# Autodesk Inventor assembly: Dedao_Mecanismo_Posição2_ComDedao
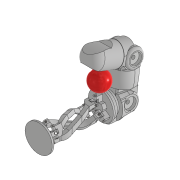
[picture p0: Inventor's stored thumbnail of the model, 180x180]
Saved by Autodesk Inventor 2020 (Build 240168000, 168)
## iProperties
Created: 2021-04-01
Part Number: Dedao_Mecanismo_Posição2_ComDedao
Document SubType Name: Assembly
Designer: deox
Author: deox
## Documents named in this file (11)
- C:\Users\deox\Desktop\TCC\Inventor Files\Dedo Kick\Dedao_Mecanismo_Posição2_ComDedao.iam
- C:\Users\deox\Desktop\TCC\Inventor Files\Dedo Kick\Base_Dedao.ipt
- C:\Users\deox\Desktop\TCC\Inventor Files\Dedo Kick\KNUCKLE_Dedao.ipt
- C:\Users\deox\Desktop\TCC\Inventor Files\Dedo Kick\LEG_Dedao.ipt
- C:\Users\deox\Desktop\TCC\Inventor Files\Dedo Kick\Pin_Dedao.ipt
- C:\Users\deox\Desktop\TCC\Inventor Files\Dedo Kick\Base_DEDAO_rot.ipt
- C:\Users\deox\Desktop\TCC\Inventor Files\Dedo Kick\Middle_DEDAO.ipt
- C:\Users\deox\Desktop\TCC\Inventor Files\Dedo Kick\ShameHider_DEDAO.ipt
- C:\Users\deox\Desktop\TCC\Inventor Files\Dedo Kick\Tip_DEDAO.ipt
- C:\Users\deox\Desktop\TCC\Inventor Files\Dedo Kick\TipTip_DEDAO.ipt
- C:\Users\deox\Desktop\TCC\Inventor Files\Dedo Kick\red_ball.ipt
## Components (29 placed, 10 different names)
1. Base_Dedao:1 — Mate:1, Mate:2, Mate:3, Mate:4, Mate:5, Mate:6, Mate:7, Mate:8, Mate:9, Mate:10, Mate:11, Mate:12, Angle:1
2. Base_Dedao:2 — Mate:25, Mate:26, Mate:27, Mate:28, Mate:29, Mate:30, Mate:31, Mate:32, Mate:33, Mate:34, Mate:35, Mate:36, Angle:1, Mate:49, Mate:50
3. KNUCKLE_Dedao:1 — Mate:9, Mate:10, Mate:13, Mate:14
4. KNUCKLE_Dedao:2 — Mate:1, Mate:2, Mate:17, Mate:18
5. KNUCKLE_Dedao:3 — Mate:5, Mate:6, Mate:21, Mate:22, Mate:60, Angle:2
6. KNUCKLE_Dedao:4 — Mate:27, Mate:28, Mate:39, Mate:40
7. KNUCKLE_Dedao:5 — Mate:25, Mate:26, Mate:37, Mate:38
8. KNUCKLE_Dedao:6 — Mate:29, Mate:30, Mate:41, Mate:42
9. LEG_Dedao:1 — Mate:13, Mate:14, Mate:15, Mate:16, Mate:37, Mate:38, Mate:47, Mate:48
10. LEG_Dedao:2 — Mate:17, Mate:18, Mate:19, Mate:20, Mate:41, Mate:42, Mate:43, Mate:44
11. LEG_Dedao:3 — Mate:21, Mate:22, Mate:23, Mate:24, Mate:39, Mate:40, Mate:45, Mate:46, Mate:60, Angle:2
12. Pin_Dedao:1 — Mate:3, Mate:4
13. Pin_Dedao:2 — Mate:11, Mate:12
14. Pin_Dedao:3 — Mate:7, Mate:8
15. Pin_Dedao:4 — Mate:19, Mate:20
16. Pin_Dedao:5 — Mate:15, Mate:16
17. Pin_Dedao:6 — Mate:23, Mate:24
18. Pin_Dedao:7 — Mate:35, Mate:36
19. Pin_Dedao:8 — Mate:33, Mate:34
20. Pin_Dedao:9 — Mate:31, Mate:32
21. Pin_Dedao:10 — Mate:43, Mate:44
22. Pin_Dedao:11 — Mate:47, Mate:48
23. Pin_Dedao:12 — Mate:45, Mate:46
24. Base_DEDAO_rot:1 — Mate:49, Mate:50, Mate:51, Mate:52
25. Middle_DEDAO:1 — Mate:51, Mate:52, Mate:53, Mate:54, Mate:55, Mate:56, Mate:57
26. ShameHider_DEDAO:1 — Mate:53, Mate:54, Mate:55
27. Tip_DEDAO:1 — Mate:56, Mate:57, Mate:58, Mate:59
28. TipTip_DEDAO:1 — Mate:58, Mate:59
29. red_ball:1
## Relationships (62: Mate 60, Angle 2)
- Mate:1: Base_Dedao:1 ↔ KNUCKLE_Dedao:2
- Mate:2: Base_Dedao:1 ↔ KNUCKLE_Dedao:2
- Mate:3: Base_Dedao:1 ↔ Pin_Dedao:1
- Mate:4: Base_Dedao:1 ↔ Pin_Dedao:1
- Mate:5: Base_Dedao:1 ↔ KNUCKLE_Dedao:3
- Mate:6: Base_Dedao:1 ↔ KNUCKLE_Dedao:3
- Mate:7: Base_Dedao:1 ↔ Pin_Dedao:3
- Mate:8: Base_Dedao:1 ↔ Pin_Dedao:3
- Mate:9: Base_Dedao:1 ↔ KNUCKLE_Dedao:1
- Mate:10: Base_Dedao:1 ↔ KNUCKLE_Dedao:1
- Mate:11: Base_Dedao:1 ↔ Pin_Dedao:2
- Mate:12: Base_Dedao:1 ↔ Pin_Dedao:2
- Mate:13: KNUCKLE_Dedao:1 ↔ LEG_Dedao:1
- Mate:14: KNUCKLE_Dedao:1 ↔ LEG_Dedao:1
- Mate:15: LEG_Dedao:1 ↔ Pin_Dedao:5
- Mate:16: LEG_Dedao:1 ↔ Pin_Dedao:5
- Mate:17: KNUCKLE_Dedao:2 ↔ LEG_Dedao:2
- Mate:18: KNUCKLE_Dedao:2 ↔ LEG_Dedao:2
- Mate:19: LEG_Dedao:2 ↔ Pin_Dedao:4
- Mate:20: LEG_Dedao:2 ↔ Pin_Dedao:4
- Mate:21: KNUCKLE_Dedao:3 ↔ LEG_Dedao:3
- Mate:22: KNUCKLE_Dedao:3 ↔ LEG_Dedao:3
- Mate:23: LEG_Dedao:3 ↔ Pin_Dedao:6
- Mate:24: LEG_Dedao:3 ↔ Pin_Dedao:6
- Mate:25: Base_Dedao:2 ↔ KNUCKLE_Dedao:5
- Mate:26: Base_Dedao:2 ↔ KNUCKLE_Dedao:5
- Mate:27: Base_Dedao:2 ↔ KNUCKLE_Dedao:4
- Mate:28: Base_Dedao:2 ↔ KNUCKLE_Dedao:4
- Mate:29: Base_Dedao:2 ↔ KNUCKLE_Dedao:6
- Mate:30: Base_Dedao:2 ↔ KNUCKLE_Dedao:6
- Mate:31: Base_Dedao:2 ↔ Pin_Dedao:9
- Mate:32: Base_Dedao:2 ↔ Pin_Dedao:9
- Mate:33: Base_Dedao:2 ↔ Pin_Dedao:8
- Mate:34: Base_Dedao:2 ↔ Pin_Dedao:8
- Mate:35: Base_Dedao:2 ↔ Pin_Dedao:7
- Mate:36: Base_Dedao:2 ↔ Pin_Dedao:7
- Mate:37: KNUCKLE_Dedao:5 ↔ LEG_Dedao:1
- Mate:38: KNUCKLE_Dedao:5 ↔ LEG_Dedao:1
- Mate:39: KNUCKLE_Dedao:4 ↔ LEG_Dedao:3
- Mate:40: KNUCKLE_Dedao:4 ↔ LEG_Dedao:3
- Mate:41: KNUCKLE_Dedao:6 ↔ LEG_Dedao:2
- Mate:42: KNUCKLE_Dedao:6 ↔ LEG_Dedao:2
- Mate:43: LEG_Dedao:2 ↔ Pin_Dedao:10
- Mate:44: LEG_Dedao:2 ↔ Pin_Dedao:10
- Mate:45: LEG_Dedao:3 ↔ Pin_Dedao:12
- Mate:46: LEG_Dedao:3 ↔ Pin_Dedao:12
- Mate:47: LEG_Dedao:1 ↔ Pin_Dedao:11
- Mate:48: LEG_Dedao:1 ↔ Pin_Dedao:11
- Angle:1 (14 deg): Base_Dedao:1 ↔ Base_Dedao:2
- Mate:49: Base_Dedao:2 ↔ Base_DEDAO_rot:1
- Mate:50: Base_Dedao:2 ↔ Base_DEDAO_rot:1
- Mate:51: Base_DEDAO_rot:1 ↔ Middle_DEDAO:1
- Mate:52: Base_DEDAO_rot:1 ↔ Middle_DEDAO:1
- Mate:53: Middle_DEDAO:1 ↔ ShameHider_DEDAO:1
- Mate:54: Middle_DEDAO:1 ↔ ShameHider_DEDAO:1
- Mate:55: Middle_DEDAO:1 ↔ ShameHider_DEDAO:1
- Mate:56: Middle_DEDAO:1 ↔ Tip_DEDAO:1
- Mate:57: Middle_DEDAO:1 ↔ Tip_DEDAO:1
- Mate:58: Tip_DEDAO:1 ↔ TipTip_DEDAO:1
- Mate:59: Tip_DEDAO:1 ↔ TipTip_DEDAO:1
- Mate:60: KNUCKLE_Dedao:3 ↔ LEG_Dedao:3
- Angle:2 (-1.99 deg): KNUCKLE_Dedao:3 ↔ LEG_Dedao:3
